# Autodesk Inventor assembly: terminal
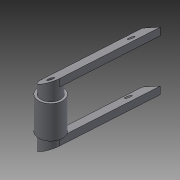
[picture p0: Inventor's stored thumbnail of the model, 180x180]
Saved by Autodesk Inventor 2018 (Build 220112000, 112)
## iProperties
Created: 2017-06-03
Part Number: terminal
Document SubType Name: Assembly
Designer: AYUSH SHUKLA
Author: AYUSH SHUKLA
## Documents named in this file (3)
- C:\Study\BTP2\Robomuse Inventor CAD\terminal.iam
- C:\Study\BTP2\Robomuse Inventor CAD\terminal.ipt
- C:\Study\BTP2\Robomuse Inventor CAD\terminal_mount.ipt
## Components (3 placed, 2 different names)
1. terminal:1 — Mate:1, Mate:2, Mate:4
2. terminal_mount:1 — Mate:1, Angle:1, Mate:3
3. terminal_mount:2 — Angle:1, Mate:2, Mate:3, Mate:4
## Relationships (5: Mate 4, Angle 1)
- Mate:1: terminal:1 ↔ terminal_mount:1
- Angle:1 (0 deg): terminal_mount:1 ↔ terminal_mount:2
- Mate:2: terminal:1 ↔ terminal_mount:2
- Mate:3 (29.3294 mm): terminal_mount:1 ↔ terminal_mount:2
- Mate:4: terminal:1 ↔ terminal_mount:2
